# Autodesk Inventor assembly: bett_V2_doppelt
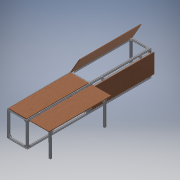
[picture p0: Inventor's stored thumbnail of the model, 180x180]
Saved by Autodesk Inventor 2018 (Build 220112000, 112)
## iProperties
Created: 2020-04-19
Part Number: bett_V2_doppelt
Material: Generisch
Document SubType Name: Assembly
Designer: wepet
Author: wepet
## Documents named in this file (5)
- C:\Users\wepet\Downloads\anhaenger\current\details\bett\bett_V2\bett_V2_doppelt.iam
- C:\Users\wepet\Downloads\anhaenger\current\details\bett\bett_V2\bett_V2_teil4_bein.iam
- C:\Users\wepet\Downloads\anhaenger\current\details\bett\bett_V2\bett_V2_teil2_deckplatte.ipt
- C:\Users\wepet\Downloads\anhaenger\current\details\bett\bett_V2\bett_V2_teil3_klappe.iam
- C:\Users\wepet\Downloads\anhaenger\current\details\bett\bett_V2\bett_V2_teil1_sitzbank.iam
## Components (10 placed, 4 different names)
1. bett_V2_teil2_deckplatte:1 — Fluchtend:1, Drehbar:2
2. bett_V2_teil3_klappe:1 [sub-assembly] — Drehbar:1, Drehbar:3, Drehbar:4
3. bett_V2_teil1_sitzbank:1 [sub-assembly] — Passend:1, Passend:2, Passend:3, Drehbar:1, Fluchtend:1, Drehbar:2, Passend:4, Fluchtend:3, Fluchtend:4
4. bett_V2_teil4_bein:1 [sub-assembly] — Drehbar:3
5. bett_V2_teil4_bein:2 [sub-assembly] — Drehbar:4
6. bett_V2_teil4_bein:3 [sub-assembly]
7. bett_V2_teil2_deckplatte:2 — Drehbar:6
8. bett_V2_teil3_klappe:2 [sub-assembly]
9. bett_V2_teil1_sitzbank:2 [sub-assembly] — Drehbar:6, Passend:4, Fluchtend:3, Fluchtend:4
10. bett_V2_teil4_bein:4 [sub-assembly]
## Relationships (16: RevoluteJoint 8, Mate 4, Flush 4)
- Passend:1 [Mate]: bett_V2_teil1_sitzbank:1
- Passend:2 [Mate]: bett_V2_teil1_sitzbank:1
- Passend:3 [Mate]: bett_V2_teil1_sitzbank:1
- Drehbar:1 [RevoluteJoint]: bett_V2_teil3_klappe:1 ↔ bett_V2_teil1_sitzbank:1
- Fluchtend:1 [Flush]: bett_V2_teil2_deckplatte:1 ↔ bett_V2_teil1_sitzbank:1
- Drehbar:2 [RevoluteJoint]: bett_V2_teil2_deckplatte:1 ↔ bett_V2_teil1_sitzbank:1
- Drehbar:3 [RevoluteJoint]: bett_V2_teil3_klappe:1 ↔ bett_V2_teil4_bein:1
- Drehbar:4 [RevoluteJoint]: bett_V2_teil3_klappe:1 ↔ bett_V2_teil4_bein:2
- [RevoluteJoint]: bett_V2_teil3_klappe:2 ↔ bett_V2_teil1_sitzbank:2
- [Flush]: bett_V2_teil2_deckplatte:2 ↔ bett_V2_teil1_sitzbank:2
- Drehbar:6 [RevoluteJoint]: bett_V2_teil2_deckplatte:2 ↔ bett_V2_teil1_sitzbank:2
- [RevoluteJoint]: bett_V2_teil4_bein:3 ↔ bett_V2_teil3_klappe:2
- [RevoluteJoint]: bett_V2_teil3_klappe:2 ↔ bett_V2_teil4_bein:4
- Passend:4 [Mate]: bett_V2_teil1_sitzbank:1 ↔ bett_V2_teil1_sitzbank:2
- Fluchtend:3 [Flush]: bett_V2_teil1_sitzbank:1 ↔ bett_V2_teil1_sitzbank:2
- Fluchtend:4 [Flush]: bett_V2_teil1_sitzbank:1 ↔ bett_V2_teil1_sitzbank:2
## Named parameters: d24_d5 = 90 deg, d25_d6 = -90 deg, d26_d7 = 0 mm, d27_d8 = 0 mm, d28_d9 = -30 deg, d29_d10 = 0 deg, d30_d11 = -90 deg, d31_d12 = 0 mm, d32_d13 = -89.373127 deg, d33_d14 = 0 deg, d34_d15 = -90 deg, d35_d20 = 0 mm, d36_d21 = -242.180958 deg, d37_d22 = -152.63 deg, d38_d23 = -242.63 deg, d39_d3 = 0 mm, d40_d4 = 90 deg
